# Autodesk Inventor assembly: WheelSuspension
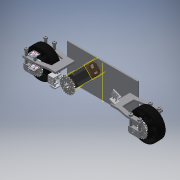
[picture p0: Inventor's stored thumbnail of the model, 180x180]
Saved by Autodesk Inventor 2017 (Build 210142000, 142)
## iProperties
Created: 2018-05-04
Part Number: WheelSuspension
Document SubType Name: Assembly
Designer: User
Author: User
## Documents named in this file (16)
- C:\Robotics\CAD\2018-19_CAD\Offseason\WheelSuspension.iam
- C:\Robotics\CAD\COTSParts\Fasteners\97345A207_316 STAINLESS STEEL SHOULDER SCREW.ipt
- C:\Robotics\CAD\COTSParts\Wheels\4in Wheel Intergreated Hub 8mm Rev2.ipt
- C:\Robotics\CAD\2016-17_CAD\Custom COTS\4inax.ipt
- C:\Robotics\CAD\2018-19_CAD\Offseason\WheelSuspensionHub.ipt
- C:\Robotics\CAD\COTSParts\Actobotics\535 parts\535198Bearing.25ID.5OD.ipt
- C:\Robotics\CAD\2018-19_CAD\Offseason\WheelandSprocketComboHub2.ipt
- C:\Robotics\CAD\COTSParts\Actobotics\615 parts\615106Sprocket.5inBore.25inPitch24Teeth.ipt
- C:\Robotics\CAD\2018-19_CAD\Offseason\WheelSuspensionFork.ipt
- C:\Robotics\CAD\2018-19_CAD\Offseason\SuspensionDrivePlate.ipt
- C:\Robotics\CAD\COTSParts\Rev\REV-41-1300HexMotor.ipt
- C:\Robotics\CAD\COTSParts\Rev\REV-41-1349HexAxle.ipt
- C:\Robotics\CAD\2018-19_CAD\Offseason\Tensioner3.iam
- C:\Robotics\CAD\COTSParts\Fasteners\91259A587_ALLOY STEEL SHOULDER SCREW.ipt
- C:\Robotics\CAD\2018-19_CAD\Offseason\Tensioner4b.iam
- C:\Robotics\CAD\2018-19_CAD\Offseason\Tensioner4a.iam
## Components (37 placed, 15 different names)
1. 4in Wheel Intergreated Hub 8mm Rev2:1 — Insert:6
2. 4inax:1 — Insert:2
3. WheelSuspensionHub:1 — Insert:1, Mate:2, Insert:10, Insert:38, Insert:39
4. 535198Bearing.25ID.5OD:1 — Insert:1, Insert:2
5. WheelandSprocketComboHub2:1 — Insert:5, Insert:6, Insert:10
6. 615106Sprocket.5inBore.25inPitch24Teeth:1 — Insert:5, Flush:29
7. WheelSuspensionHub:2 — Insert:7, Insert:37, Insert:40
8. 535198Bearing.25ID.5OD:2 — Insert:7, Mate:2
9. WheelSuspensionFork:1 — Angle:1, Insert:27, Insert:28, Insert:31, Insert:34, Mate:47, Mate:48, Mate:49, Insert:36
10. 97345A207_316 STAINLESS STEEL SHOULDER SCREW:5
11. 4in Wheel Intergreated Hub 8mm Rev2:2
12. 4inax:2 — Mate:22
13. WheelSuspensionHub:3
14. 535198Bearing.25ID.5OD:3
15. WheelandSprocketComboHub2:2 — Mate:22, Insert:35
16. 615106Sprocket.5inBore.25inPitch24Teeth:2 — Flush:27
17. WheelSuspensionHub:4 — Insert:35
18. 97345A207_316 STAINLESS STEEL SHOULDER SCREW:6
19. 535198Bearing.25ID.5OD:4
20. WheelSuspensionFork:2 — Insert:29, Insert:30, Insert:32, Insert:33
21. 97345A207_316 STAINLESS STEEL SHOULDER SCREW:7
22. 97345A207_316 STAINLESS STEEL SHOULDER SCREW:8
23. SuspensionDrivePlate:1 — Insert:27, Insert:28, Insert:29, Insert:30, Mate:23, Mate:30, Mate:31, Mate:50, Flush:30, Mate:51, Flush:31
24. SuspensionDrivePlate:2 — Insert:31, Insert:32, Insert:33, Insert:34, Mate:6, Flush:1, Flush:2, Mate:27, Mate:28, Flush:24, Angle:6, Angle:8, Mate:36, Mate:37, Mate:38, Mate:53
25. REV-41-1300HexMotor:1 — Mate:14, Flush:5, Angle:2, Mate:27, Mate:28, Flush:24
26. REV-41-1349HexAxle:2 — Mate:14, Flush:5, Angle:2, Mate:35
27. Tensioner3:1 [sub-assembly] — Mate:23, Mate:30, Mate:31, Angle:6
28. 615106Sprocket.5inBore.25inPitch24Teeth:4 — Mate:35, Flush:27
29. REV-41-1300HexMotor:2 — Angle:8, Mate:36, Mate:37, Mate:38, Mate:39, Mate:40, Flush:28
30. 615106Sprocket.5inBore.25inPitch24Teeth:5 — Mate:41, Flush:29
31. REV-41-1349HexAxle:3 — Mate:39, Mate:40, Flush:28, Mate:41
32. 91259A587_ALLOY STEEL SHOULDER SCREW:1 — Mate:47, Insert:39
33. 91259A587_ALLOY STEEL SHOULDER SCREW:2 — Mate:48, Insert:37
34. 91259A587_ALLOY STEEL SHOULDER SCREW:3 — Mate:49, Insert:40
35. 91259A587_ALLOY STEEL SHOULDER SCREW:4 — Insert:36, Insert:38
36. Tensioner4b:1 [sub-assembly] — Mate:51, Mate:52, Flush:31
37. Tensioner4a:1 [sub-assembly] — Mate:50, Flush:30, Mate:52, Mate:53
## Relationships (69: Insert 31, Mate 25, Flush 9, Angle 4)
- Insert:1: WheelSuspensionHub:1 ↔ 535198Bearing.25ID.5OD:1
- Insert:2 (3.175 mm): 4inax:1 ↔ 535198Bearing.25ID.5OD:1
- Insert:5: WheelandSprocketComboHub2:1 ↔ 615106Sprocket.5inBore.25inPitch24Teeth:1
- Insert:6: 4in Wheel Intergreated Hub 8mm Rev2:1 ↔ WheelandSprocketComboHub2:1
- Insert:7: WheelSuspensionHub:2 ↔ 535198Bearing.25ID.5OD:2
- Mate:2: WheelSuspensionHub:1 ↔ 535198Bearing.25ID.5OD:2
- Angle:1 (0 deg): WheelSuspensionFork:1
- Insert:10 (1.27 mm): WheelSuspensionHub:1 ↔ WheelandSprocketComboHub2:1
- [Insert]: WheelSuspensionHub:3 ↔ 535198Bearing.25ID.5OD:3
- [Insert] (3.175 mm): 4inax:2 ↔ 535198Bearing.25ID.5OD:3
- [Insert]: 97345A207_316 STAINLESS STEEL SHOULDER SCREW:5 ↔ WheelSuspensionHub:3
- [Insert]: WheelandSprocketComboHub2:2 ↔ 615106Sprocket.5inBore.25inPitch24Teeth:2
- [Insert]: 4in Wheel Intergreated Hub 8mm Rev2:2 ↔ WheelandSprocketComboHub2:2
- [Insert]: WheelSuspensionHub:4 ↔ 535198Bearing.25ID.5OD:4
- [Insert]: WheelSuspensionHub:4 ↔ 97345A207_316 STAINLESS STEEL SHOULDER SCREW:6
- [Mate]: WheelSuspensionHub:3 ↔ 535198Bearing.25ID.5OD:4
- [Mate] (63.5 mm): 97345A207_316 STAINLESS STEEL SHOULDER SCREW:5 ↔ 97345A207_316 STAINLESS STEEL SHOULDER SCREW:6
- [Insert]: 97345A207_316 STAINLESS STEEL SHOULDER SCREW:5 ↔ WheelSuspensionFork:2
- [Insert]: 97345A207_316 STAINLESS STEEL SHOULDER SCREW:6 ↔ WheelSuspensionFork:2
- [Insert]: WheelSuspensionFork:2 ↔ 97345A207_316 STAINLESS STEEL SHOULDER SCREW:7
- [Insert]: WheelSuspensionFork:2 ↔ 97345A207_316 STAINLESS STEEL SHOULDER SCREW:8
- Insert:27: WheelSuspensionFork:1 ↔ SuspensionDrivePlate:1
- Insert:28: WheelSuspensionFork:1 ↔ SuspensionDrivePlate:1
- Insert:29: WheelSuspensionFork:2 ↔ SuspensionDrivePlate:1
- Insert:30: WheelSuspensionFork:2 ↔ SuspensionDrivePlate:1
- Insert:31: WheelSuspensionFork:1 ↔ SuspensionDrivePlate:2
- Insert:32: WheelSuspensionFork:2 ↔ SuspensionDrivePlate:2
- Insert:33: WheelSuspensionFork:2 ↔ SuspensionDrivePlate:2
- Insert:34: WheelSuspensionFork:1 ↔ SuspensionDrivePlate:2
- Mate:6: SuspensionDrivePlate:2
- Flush:1: SuspensionDrivePlate:2
- Flush:2: SuspensionDrivePlate:2
- Mate:14: REV-41-1300HexMotor:1 ↔ REV-41-1349HexAxle:2
- Flush:5 (-25.4 mm): REV-41-1300HexMotor:1 ↔ REV-41-1349HexAxle:2
- Angle:2 (0 deg): REV-41-1300HexMotor:1 ↔ REV-41-1349HexAxle:2
- Mate:22: 4inax:2 ↔ WheelandSprocketComboHub2:2
- Mate:23: SuspensionDrivePlate:1 ↔ Tensioner3:1
- Mate:27: SuspensionDrivePlate:2 ↔ REV-41-1300HexMotor:1
- Mate:28 (-3.175 mm): SuspensionDrivePlate:2 ↔ REV-41-1300HexMotor:1
- Flush:24 (12.7 mm): SuspensionDrivePlate:2 ↔ REV-41-1300HexMotor:1
- Mate:30: SuspensionDrivePlate:1 ↔ Tensioner3:1
- Mate:31: SuspensionDrivePlate:1 ↔ Tensioner3:1
- Angle:6 (21.8 deg): SuspensionDrivePlate:2 ↔ Tensioner3:1
- Mate:35: REV-41-1349HexAxle:2 ↔ 615106Sprocket.5inBore.25inPitch24Teeth:4
- Flush:27: 615106Sprocket.5inBore.25inPitch24Teeth:2 ↔ 615106Sprocket.5inBore.25inPitch24Teeth:4
- Insert:35 (1.27 mm): WheelandSprocketComboHub2:2 ↔ WheelSuspensionHub:4
- Angle:8 (135 deg): SuspensionDrivePlate:2 ↔ REV-41-1300HexMotor:2
- Mate:36 (-34.925 mm): SuspensionDrivePlate:2 ↔ REV-41-1300HexMotor:2
- Mate:37: SuspensionDrivePlate:2 ↔ REV-41-1300HexMotor:2
- Mate:38 (-50.8 mm): SuspensionDrivePlate:2 ↔ REV-41-1300HexMotor:2
- Mate:39: REV-41-1300HexMotor:2 ↔ REV-41-1349HexAxle:3
- Mate:40: REV-41-1300HexMotor:2 ↔ REV-41-1349HexAxle:3
- Flush:28 (-25.4 mm): REV-41-1300HexMotor:2 ↔ REV-41-1349HexAxle:3
- Mate:41: 615106Sprocket.5inBore.25inPitch24Teeth:5 ↔ REV-41-1349HexAxle:3
- Flush:29: 615106Sprocket.5inBore.25inPitch24Teeth:1 ↔ 615106Sprocket.5inBore.25inPitch24Teeth:5
- Mate:47: WheelSuspensionFork:1 ↔ 91259A587_ALLOY STEEL SHOULDER SCREW:1
- Mate:48: WheelSuspensionFork:1 ↔ 91259A587_ALLOY STEEL SHOULDER SCREW:2
- Mate:49: WheelSuspensionFork:1 ↔ 91259A587_ALLOY STEEL SHOULDER SCREW:3
- Insert:36 (15.875 mm): WheelSuspensionFork:1 ↔ 91259A587_ALLOY STEEL SHOULDER SCREW:4
- Insert:37: WheelSuspensionHub:2 ↔ 91259A587_ALLOY STEEL SHOULDER SCREW:2
- Insert:38: WheelSuspensionHub:1 ↔ 91259A587_ALLOY STEEL SHOULDER SCREW:4
- Insert:39: WheelSuspensionHub:1 ↔ 91259A587_ALLOY STEEL SHOULDER SCREW:1
- Insert:40: WheelSuspensionHub:2 ↔ 91259A587_ALLOY STEEL SHOULDER SCREW:3
- Mate:50: SuspensionDrivePlate:1 ↔ Tensioner4a:1
- Flush:30: SuspensionDrivePlate:1 ↔ Tensioner4a:1
- Mate:51: SuspensionDrivePlate:1 ↔ Tensioner4b:1
- Mate:52: Tensioner4b:1 ↔ Tensioner4a:1
- Flush:31: SuspensionDrivePlate:1 ↔ Tensioner4b:1
- Mate:53 (-34.925 mm): SuspensionDrivePlate:2 ↔ Tensioner4a:1
## Named parameters: d23_d18 = 0 mm, d24_d19 = 0 mm, d25_d20 = 0 mm, d26_d21 = 0 mm, d27_d0 = 0 mm, d28_d1 = 3.175 mm, d29_d2 = 0 mm, d30_d5 = 0 mm, d31_d6 = 0 mm, d32_d7 = 0 mm, d33_d9 = 0 mm, d34_d12 = 0 mm, d35_d14 = 63.5 mm
